# Autodesk Inventor assembly: body
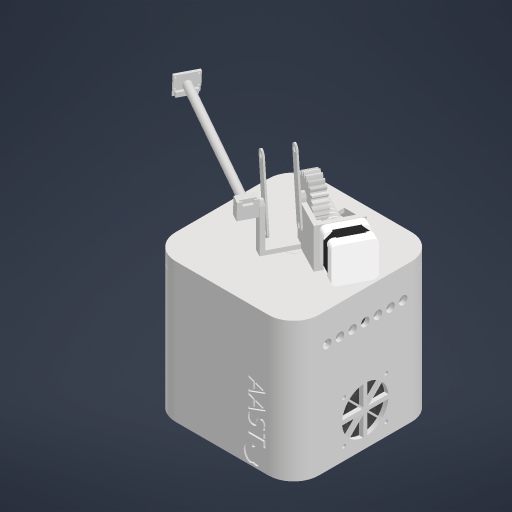
[picture p0: Inventor's stored thumbnail of the model, 512x512]
Saved by Autodesk Inventor 2024 (Build 280153000, 153)
## iProperties
Created: 2023-06-18
Part Number: body
Document SubType Name: Assembly
Designer: 6gioc
Author: 6gioc
## Documents named in this file (9)
- C:\Users\6gioc\OneDrive\AAST\PART\body.iam
- C:\Users\6gioc\OneDrive\AAST\PART\bottom case.ipt
- C:\Users\6gioc\OneDrive\AAST\PART\top.ipt
- C:\Users\6gioc\OneDrive\AAST\PART\gun assemble v1.iam
- C:\Users\6gioc\OneDrive\AAST\PART\m10 tube.ipt
- C:\Users\6gioc\OneDrive\AAST\PART\stepmotor v1.ipt
- C:\Users\6gioc\OneDrive\AAST\PART\worm.iam
- C:\Users\6gioc\OneDrive\AAST\PART\Fan 60x60x25mm\Fan 60x60x25mm.iam
- C:\Users\6gioc\OneDrive\AAST\PART\40mm_gear_hexagon.iam
## Components (9 placed, 8 different names)
1. bottom case:1 — 강체:1, 강체:3, 강체:4
2. top:1 — 강체:1, 회전:1, 회전:2, 강체:2, 회전:4, 회전:6
3. gun assemble v1:1 [sub-assembly] — 회전:1, 강체:5
4. m10 tube:1 — 회전:2
5. stepmotor v1:1 — 강체:2, 회전:4, 회전:5, 회전:6
6. worm:1 [sub-assembly] — 회전:5, 회전:1
7. Fan 60x60x25mm:1 [sub-assembly] — 강체:4
8. Fan 60x60x25mm:2 [sub-assembly] — 강체:3
9. 40mm_gear_hexagon:1 [sub-assembly] — 강체:5, 회전:1
## Relationships (11: WeldJoint 5, RevoluteJoint 5, RelateRotation 1)
- 강체:1 [WeldJoint]: bottom case:1 ↔ top:1
- 회전:1 [RevoluteJoint]: top:1 ↔ gun assemble v1:1
- 회전:2 [RevoluteJoint]: top:1 ↔ m10 tube:1
- 강체:2 [WeldJoint]: top:1 ↔ stepmotor v1:1
- 회전:4 [RevoluteJoint]: top:1 ↔ stepmotor v1:1
- 회전:5 [RevoluteJoint] (-15 mm): stepmotor v1:1 ↔ worm:1
- 회전:6 [RevoluteJoint]: top:1 ↔ stepmotor v1:1
- 강체:3 [WeldJoint]: bottom case:1 ↔ Fan 60x60x25mm:2
- 강체:4 [WeldJoint]: bottom case:1 ↔ Fan 60x60x25mm:1
- 강체:5 [WeldJoint]: gun assemble v1:1 ↔ 40mm_gear_hexagon:1
- 회전:1 [RelateRotation] (20 ul): worm:1 ↔ 40mm_gear_hexagon:1
